# Autodesk Inventor assembly: turret assembly
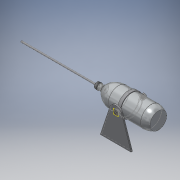
[picture p0: Inventor's stored thumbnail of the model, 180x180]
Saved by Autodesk Inventor 2019 (Build 230136000, 136)
## iProperties
Created: 2022-03-28
Part Number: turret assembly
Document SubType Name: Assembly
Designer: Ian
Author: Ian
## Documents named in this file (7)
- D:\Ian\Documents\Projects\autoturret\mechanical design\turret assembly.iam
- D:\Ian\Documents\Projects\autoturret\mechanical design\norm bottle.iam
- D:\Ian\Documents\Projects\autoturret\mechanical design\brake line.ipt
- D:\Ian\Documents\Projects\autoturret\mechanical design\bottle clamp.ipt
- D:\Ian\Documents\Projects\autoturret\mechanical design\wierd bearing interface part.ipt
- D:\Ian\Documents\Projects\autoturret\mechanical design\608 skate bearing.ipt
- D:\Ian\Documents\Projects\autoturret\mechanical design\left stand.ipt
## Components (8 placed, 6 different names)
1. norm bottle:1 [sub-assembly] — Insert:1
2. brake line:1 — Insert:1
3. bottle clamp:1 — Flush:1, Mate:1, Flush:2, Mate:2, Flush:3, Flush:4
4. wierd bearing interface part:1 — Flush:1, Mate:1, Flush:2, Insert:2
5. wierd bearing interface part:2 — Mate:2, Flush:3, Flush:4, Insert:3
6. 608 skate bearing:1 — Insert:3
7. 608 skate bearing:2 — Insert:2, Flush:5, Flush:6
8. left stand:1 — Flush:5, Flush:6
## Relationships (11: Flush 6, Insert 3, Mate 2)
- Insert:1 (-40 mm): norm bottle:1 ↔ brake line:1
- Flush:1: bottle clamp:1 ↔ wierd bearing interface part:1
- Mate:1 (2 mm): bottle clamp:1 ↔ wierd bearing interface part:1
- Flush:2: bottle clamp:1 ↔ wierd bearing interface part:1
- Mate:2 (2 mm): bottle clamp:1 ↔ wierd bearing interface part:2
- Flush:3: bottle clamp:1 ↔ wierd bearing interface part:2
- Flush:4: bottle clamp:1 ↔ wierd bearing interface part:2
- Insert:2: wierd bearing interface part:1 ↔ 608 skate bearing:2
- Insert:3: wierd bearing interface part:2 ↔ 608 skate bearing:1
- Flush:5: 608 skate bearing:2 ↔ left stand:1
- Flush:6: 608 skate bearing:2 ↔ left stand:1
